# Autodesk Inventor assembly: 頭
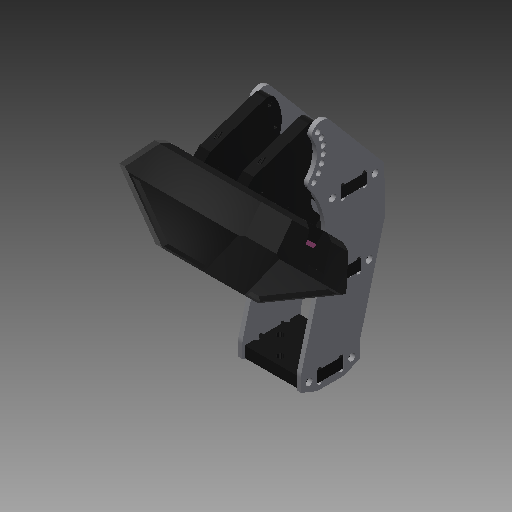
[picture p0: Inventor's stored thumbnail of the model, 512x512]
Saved by Autodesk Inventor 2018 (Build 220112000, 112)
## iProperties
Created: 2018-06-08
Part Number: 頭
Material: 一般
Document SubType Name: Assembly
Designer: taka
Mass: 102.797 g
Surface Area: 498.656 cm^2
Volume: 92.836 cm^3
Density: 1.1073 g/cm^3
Author: taka
## Documents named in this file (8)
- C:\Users\taka\Documents\git\OpenPlatform\mechanism\OpenPlatform_ver3_0\上半身\頭\頭.iam
- C:\Users\taka\Documents\git\OpenPlatform\mechanism\OpenPlatform_ver3_0\上半身\頭\頭_メインフレーム.ipt
- C:\Users\taka\Documents\git\OpenPlatform\mechanism\OpenPlatform_ver3_0\上半身\頭\頭_サブフレーム.ipt
- C:\Users\taka\Documents\git\OpenPlatform\mechanism\OpenPlatform_ver3_0\上半身\頭\頭_サーボホーンフレーム.ipt
- C:\Users\taka\Documents\git\OpenPlatform\mechanism\OpenPlatform_ver3_0\上半身\頭\カメラ_メインフレーム.ipt
- C:\Users\taka\Documents\git\OpenPlatform\mechanism\OpenPlatform_ver3_0\上半身\頭\カメラ_メインフレーム1_KBCR-S02MU.ipt
- C:\Users\taka\Documents\git\OpenPlatform\mechanism\OpenPlatform_ver3_0\上半身\頭\KBCR-S02MU.ipt
- C:\Users\taka\Documents\git\OpenPlatform\mechanism\OpenPlatform_ver3_0\上半身\頭\カメラ_外装.ipt
## Components (10 placed, 7 different names)
1. 頭_メインフレーム:1 — 挿入:1, 挿入:5, 挿入:6, 挿入:8, 挿入:22, 挿入:23
2. 頭_メインフレーム:2 — 挿入:2, 挿入:3, 挿入:4, 挿入:7, 挿入:17, 挿入:18
3. 頭_サブフレーム:1 — 挿入:1, 挿入:2, 挿入:4
4. 頭_サブフレーム:2 — 挿入:3, 挿入:5, 挿入:6
5. 頭_サーボホーンフレーム:1 — 挿入:7, 挿入:8
6. カメラ_メインフレーム:1 — 挿入:22, 挿入:23, 挿入:25
7. カメラ_メインフレーム:2 — 挿入:17, 挿入:18, 挿入:24
8. カメラ_メインフレーム1_KBCR-S02MU:1 — 挿入:24, 挿入:25, 挿入:26, 挿入:27, 挿入:28, 正接:1
9. KBCR-S02MU:1 — 挿入:26, 挿入:27
10. カメラ_外装:1 — 挿入:28, 正接:1
## Relationships (18: Insert 17, Tangent 1)
- 挿入:1 [Insert]: 頭_メインフレーム:1 ↔ 頭_サブフレーム:1
- 挿入:2 [Insert]: 頭_メインフレーム:2 ↔ 頭_サブフレーム:1
- 挿入:3 [Insert]: 頭_メインフレーム:2 ↔ 頭_サブフレーム:2
- 挿入:4 [Insert]: 頭_メインフレーム:2 ↔ 頭_サブフレーム:1
- 挿入:5 [Insert]: 頭_メインフレーム:1 ↔ 頭_サブフレーム:2
- 挿入:6 [Insert]: 頭_メインフレーム:1 ↔ 頭_サブフレーム:2
- 挿入:7 [Insert]: 頭_メインフレーム:2 ↔ 頭_サーボホーンフレーム:1
- 挿入:8 [Insert]: 頭_メインフレーム:1 ↔ 頭_サーボホーンフレーム:1
- 挿入:17 [Insert]: 頭_メインフレーム:2 ↔ カメラ_メインフレーム:2
- 挿入:18 [Insert]: 頭_メインフレーム:2 ↔ カメラ_メインフレーム:2
- 挿入:22 [Insert]: 頭_メインフレーム:1 ↔ カメラ_メインフレーム:1
- 挿入:23 [Insert]: 頭_メインフレーム:1 ↔ カメラ_メインフレーム:1
- 挿入:24 [Insert]: カメラ_メインフレーム:2 ↔ カメラ_メインフレーム1_KBCR-S02MU:1
- 挿入:25 [Insert]: カメラ_メインフレーム:1 ↔ カメラ_メインフレーム1_KBCR-S02MU:1
- 挿入:26 [Insert]: カメラ_メインフレーム1_KBCR-S02MU:1 ↔ KBCR-S02MU:1
- 挿入:27 [Insert]: カメラ_メインフレーム1_KBCR-S02MU:1 ↔ KBCR-S02MU:1
- 挿入:28 [Insert]: カメラ_メインフレーム1_KBCR-S02MU:1 ↔ カメラ_外装:1
- 正接:1 [Tangent]: カメラ_メインフレーム1_KBCR-S02MU:1 ↔ カメラ_外装:1
